# Autodesk Inventor assembly: Base
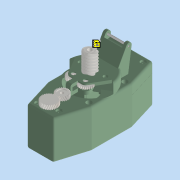
[picture p0: Inventor's stored thumbnail of the model, 180x180]
Saved by Autodesk Inventor 2020.2 (Build 242310000, 310)
## iProperties
Created: 2020-03-15
Part Number: Base
Document SubType Name: Assembly
Designer: JochenAlt
Author: JochenAlt
## Documents named in this file (6)
- D:\Projects\MiniBot\CAD\gripper\Base.iam
- D:\Projects\MiniBot\CAD\gripper\Base.ipt
- D:\Projects\MiniBot\CAD\gripper\Base\Konstruktions-Assistent\KnuckleGear.iam
- D:\Projects\MiniBot\CAD\WristGear\Konstruktions-Assistent\Stirnräder2.iam
- D:\Projects\MiniBot\CAD\gripper\Base\Konstruktions-Assistent\Schneckenräder1.iam
- D:\Projects\MiniBot\CAD\gripper\Base\Konstruktions-Assistent\Stirnräder1.iam
## Components (5 placed, 3 different names)
1. Base:1 — Passend:1, Passend:4
2. Stirnräder:1 [sub-assembly] — Passend:1
3. Stirnräder:2 [sub-assembly] — Passend:4
4. Schneckenräder:1 [sub-assembly]
5. Stirnräder:3 [sub-assembly]
## Relationships (2: Mate 2)
- Passend:1 [Mate]: Base:1 ↔ Stirnräder:1
- Passend:4 [Mate]: Base:1 ↔ Stirnräder:2
